# Autodesk Inventor assembly: subsystem1
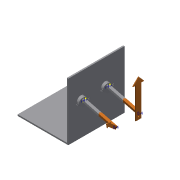
[picture p0: Inventor's stored thumbnail of the model, 180x180]
Saved by Autodesk Inventor 2019 (Build 230136000, 136)
## iProperties
Created: 2019-12-09
Part Number: subsystem1
Document SubType Name: Assembly
Designer: Abhishek
Author: Abhishek
## Documents named in this file (4)
- E:\subsystem1.iam
- E:\shafthold.iam
- E:\needle.ipt
- E:\lateneedle.ipt
## Components (3 placed, 3 different names)
1. shafthold:1 [sub-assembly] — Mate:1, Rigid:1
2. needle:1 — Mate:1
3. lateneedle:1 — Rigid:1
## Relationships (2: Mate 1, WeldJoint 1)
- Mate:1: shafthold:1 ↔ needle:1
- Rigid:1 [WeldJoint]: shafthold:1 ↔ lateneedle:1
